# Autodesk Inventor assembly: onderkant
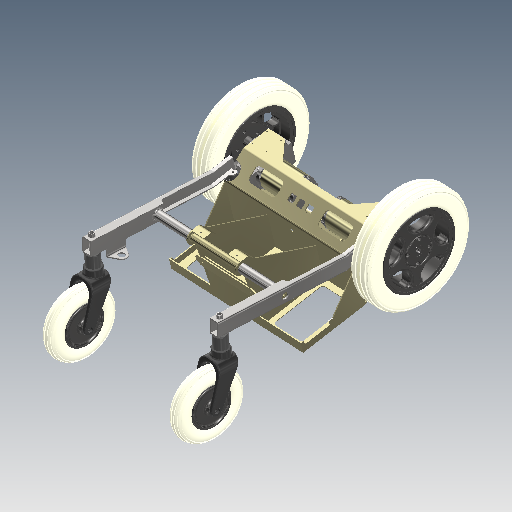
[picture p0: Inventor's stored thumbnail of the model, 512x512]
Saved by Autodesk Inventor 2020.3 (Build 243373000, 373)
## iProperties
Created: 2020-09-17
Part Number: onderkant
Document SubType Name: Assembly
Designer: Svend
Author: Svend
## Documents named in this file (13)
- C:\Users\Svend\OneDrive\Documents\GitHub\Rolstoel\onderkant.iam
- C:\Users\Svend\OneDrive\Documents\GitHub\Rolstoel\frame onderkant.ipt
- C:\Users\Svend\OneDrive\Documents\GitHub\Rolstoel\achterwiel.iam
- C:\Users\Svend\OneDrive\Documents\GitHub\Rolstoel\rubber.ipt
- C:\Users\Svend\OneDrive\Documents\GitHub\Rolstoel\balk.ipt
- C:\Users\Svend\OneDrive\Documents\GitHub\Rolstoel\wielhub.ipt
- C:\Users\Svend\OneDrive\Documents\GitHub\Rolstoel\ring wiel.ipt
- C:\Users\Svend\OneDrive\Documents\GitHub\Rolstoel\velg.ipt
- C:\Users\Svend\OneDrive\Documents\GitHub\Rolstoel\motor.ipt
- C:\Users\Svend\OneDrive\Documents\GitHub\Rolstoel\motor rechts.ipt
- C:\Users\Svend\OneDrive\Documents\GitHub\Rolstoel\bodum.ipt
- C:\Users\Svend\OneDrive\Documents\GitHub\Rolstoel\frame onderkant rechts v2.ipt
- C:\Users\Svend\OneDrive\Documents\GitHub\Rolstoel\spacerwiel.ipt
## Components (18 placed, 12 different names)
1. frame onderkant rechts v2:1 — Mate:2, Mate:3, Mate:4, Mate:32, Mate:33
2. frame onderkant:1 — Mate:1, Mate:3, Mate:4, Mate:5, Mate:6, Mate:29, Mate:30, Mate:31
3. achterwiel:1 [sub-assembly] — Mate:1, Flush:1, Mate:5, Mate:35, Mate:36
4. achterwiel:2 [sub-assembly] — Mate:2, Flush:1, Mate:37, Mate:38
5. rubber:1 — Mate:6, Mate:11, Mate:12, Mate:31
6. rubber:2 — Mate:10, Mate:32, Mate:33
7. balk:1 — Mate:10, Mate:11, Mate:12, Flush:4, Mate:34
8. wielhub:1 — Mate:13, Mate:14, Mate:15, Mate:16, Mate:17, Mate:24, Mate:28, Flush:4
9. ring wiel:1 — Mate:16, Mate:17, Mate:25
10. velg:1 — Mate:13, Mate:14, Mate:15, Mate:27
11. wielhub:2 — Mate:23, Mate:28
12. ring wiel:2 — Mate:26
13. velg:2 — Mate:27
14. motor:1 — Mate:24, Mate:25, Flush:2, Flush:3, Mate:34
15. motor rechts:1 — Mate:23, Mate:26, Flush:2, Flush:3, Angle:1
16. bodum:1 — Mate:29, Mate:30, Angle:1
17. spacerwiel:1 — Mate:35, Mate:36
18. spacerwiel:2 — Mate:37, Mate:38
## Relationships (40: Mate 35, Flush 4, Angle 1)
- Mate:1: frame onderkant:1 ↔ achterwiel:1
- Mate:2: frame onderkant rechts v2:1 ↔ achterwiel:2
- Mate:3: frame onderkant rechts v2:1 ↔ frame onderkant:1
- Flush:1: achterwiel:1 ↔ achterwiel:2
- Mate:4 (-470 mm): frame onderkant rechts v2:1 ↔ frame onderkant:1
- Mate:5 (40 mm): frame onderkant:1 ↔ achterwiel:1
- Mate:6: frame onderkant:1 ↔ rubber:1
- Mate:10: rubber:2 ↔ balk:1
- Mate:11: rubber:1 ↔ balk:1
- Mate:12: rubber:1 ↔ balk:1
- Mate:13: wielhub:1 ↔ velg:1
- Mate:14: wielhub:1 ↔ velg:1
- Mate:15: wielhub:1 ↔ velg:1
- Mate:16: wielhub:1 ↔ ring wiel:1
- Mate:17: wielhub:1 ↔ ring wiel:1
- [Mate]: wielhub:2 ↔ velg:2
- [Mate]: wielhub:2 ↔ velg:2
- [Mate]: wielhub:2 ↔ velg:2
- [Mate]: wielhub:2 ↔ ring wiel:2
- [Mate]: wielhub:2 ↔ ring wiel:2
- Mate:23: wielhub:2 ↔ motor rechts:1
- Mate:24: wielhub:1 ↔ motor:1
- Mate:25: ring wiel:1 ↔ motor:1
- Mate:26: ring wiel:2 ↔ motor rechts:1
- Mate:27: velg:1 ↔ velg:2
- Flush:2: motor:1 ↔ motor rechts:1
- Flush:3: motor:1 ↔ motor rechts:1
- Mate:28 (-610 mm): wielhub:1 ↔ wielhub:2
- Flush:4 (305 mm): balk:1 ↔ wielhub:1
- Mate:29: frame onderkant:1 ↔ bodum:1
- Mate:30: frame onderkant:1 ↔ bodum:1
- Angle:1 (0 deg): motor rechts:1 ↔ bodum:1
- Mate:31: frame onderkant:1 ↔ rubber:1
- Mate:32: frame onderkant rechts v2:1 ↔ rubber:2
- Mate:33: frame onderkant rechts v2:1 ↔ rubber:2
- Mate:34 (10 mm): balk:1 ↔ motor:1
- Mate:35: achterwiel:1 ↔ spacerwiel:1
- Mate:36: achterwiel:1 ↔ spacerwiel:1
- Mate:37: achterwiel:2 ↔ spacerwiel:2
- Mate:38: achterwiel:2 ↔ spacerwiel:2
## Named parameters: d20_d15 = 0 mm, d21_d16 = 0 mm, d22_d17 = 0 mm, d23_d18 = 0 mm, d24_d19 = 0 mm
